# Autodesk Inventor assembly: Collector Assembly V2
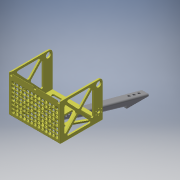
[picture p0: Inventor's stored thumbnail of the model, 180x180]
Saved by Autodesk Inventor 2019 (Build 230136000, 136)
## iProperties
Created: 2019-01-31
Part Number: Collector Assembly V2
Document SubType Name: Assembly
Designer: Ashley
Author: Ashley
## Documents named in this file (3)
- C:\Users\Ashley\Desktop\repositories\design\inventor\2018-2019\Collector Rendition 2.0\Collector Assembly V2.iam
- C:\Users\Ashley\Desktop\repositories\design\inventor\2018-2019\Collector Rendition 2.0\Collector V2.ipt
- C:\Users\Ashley\Desktop\repositories\design\inventor\2018-2019\Collector Rendition 2.0\Rev Xrail attatchment.ipt
## Components (2 placed, 2 different names)
1. Collector V2:1 — Insert:1
2. Rev Xrail attatchment:1 — Insert:1
## Relationships (1: Insert 1)
- Insert:1: Collector V2:1 ↔ Rev Xrail attatchment:1
